# Autodesk Inventor assembly: Assembly
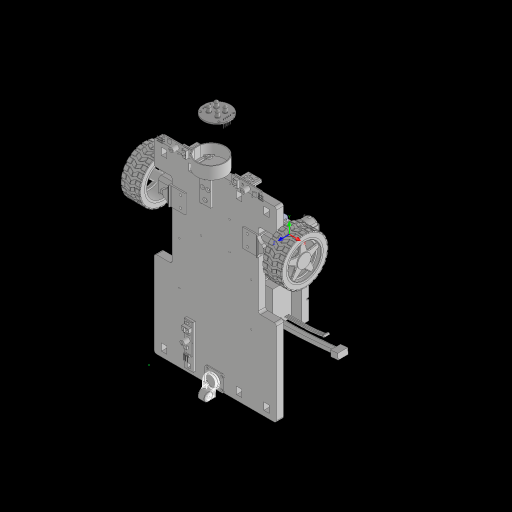
[picture p0: Inventor's stored thumbnail of the model, 512x512]
Saved by Autodesk Inventor 2024.3 (Build 283343010, 343A)
## iProperties
Created: 2025-04-09
Part Number: Assembly
Document SubType Name: Assembly
Designer: Oleg Kelner
Author: Oleg Kelner
## Documents named in this file (21)
- D:\Study\Prototyping\Prototyping-SS25-Team-C4\3DModels\Assembly.iam
- D:\Study\Prototyping\Prototyping-SS25-Team-C4\3DModels\Basic components\chassis.ipt
- D:\Study\Prototyping\Prototyping-SS25-Team-C4\3DModels\Basic components\motor-with-tire.ipt
- D:\Study\Prototyping\Prototyping-SS25-Team-C4\3DModels\Basic components\front-wheel.ipt
- D:\Study\Prototyping\Prototyping-SS25-Team-C4\3DModels\Basic components\motor-with-tire_MIR.ipt
- D:\Study\Prototyping\Prototyping-SS25-Team-C4\3DModels\Basic components\lipo-battery.ipt
- D:\Study\Prototyping\Prototyping-SS25-Team-C4\3DModels\Basic components\arduino.ipt
- D:\Study\Prototyping\Prototyping-SS25-Team-C4\3DModels\Basic components\breadboard.ipt
- D:\Study\Prototyping\Prototyping-SS25-Team-C4\3DModels\Basic components\motorcontroler.ipt
- D:\Study\Prototyping\Prototyping-SS25-Team-C4\3DModels\Details to print\.ipt\vertMotorHolder.ipt
- D:\Study\Prototyping\Prototyping-SS25-Team-C4\3DModels\Details to print\.ipt\batteryHolder.ipt
- D:\Work\HSHL\Kart\Kart Assembly Parts\infrared-sensor-new.ipt
- D:\Study\Prototyping\Prototyping-SS25-Team-C4\3DModels\Details to print\.ipt\IRsensorHolder.ipt
- D:\Study\Prototyping\Prototyping-SS25-Team-C4\3DModels\Details to print\.ipt\IRsensorHolder2.ipt
- D:\Work\HSHL\Kart\Kart Assembly Parts\ultrasonic-sensor.ipt
- D:\Work\HSHL\Kart\Kart Assembly Parts\ColourSensor.ipt
- D:\Study\Prototyping\Prototyping-SS25-Team-C4\3DModels\Details to print\.ipt\ultrasomicHolder.ipt
- D:\Study\Prototyping\Prototyping-SS25-Team-C4\3DModels\Details to print\.ipt\IRHolder_new.ipt
- D:\Study\Prototyping\Prototyping-SS25-Team-C4\3DModels\Details to print\.ipt\IRHolder_new2.ipt
- D:\Study\Prototyping\Prototyping-SS25-Team-C4\3DModels\Details to print\.ipt\colorSensorHolder.ipt
- D:\Study\Prototyping\Prototyping-SS25-Team-C4\3DModels\Details to print\.ipt\colorSensorHolder2.ipt
## Components (26 placed, 20 different names)
1. chassis:1 — Rigid:1, Rigid:2, Rigid:3, Slider:1, Angle:1, Mate:1, Flush:2, Mate:3, Flush:5, Flush:6, Planar:2, Angle:2, Planar:3, Flush:8, Angle:3, Flush:10, Flush:14, Flush:15, Flush:16, Flush:18
2. motor-with-tire:1 — Rotational:11, Rotational:12, Tangent:1
3. front-wheel:1 — Rigid:1
4. motor-with-tire_MIR:1 — Rotational:9, Rotational:10
5. lipo-battery:1 — Slider:1, Rigid:4, Rigid:5, Rigid:6
6. arduino:1 — Planar:2, Angle:2
7. breadboard:1 — Rigid:5
8. motorcontroler:1 — Planar:3, Flush:7, Flush:8
9. vertMotorHolder:1 — Rigid:3, Mate:2, Rotational:11, Rotational:12, Flush:7
10. vertMotorHolder:2 — Rigid:2, Rotational:9, Rotational:10
11. batteryHolder:1 — Mate:2, Rigid:4
12. batteryHolder:2 — Rigid:6
13. infrared-sensor-new:1 — Rotational:5, Rotational:6, Flush:9
14. IRsensorHolder:1 — Angle:1, Rotational:5, Rotational:6, Mate:4, Flush:11
15. IRsensorHolder2:1 — Mate:1, Flush:2, Flush:10, Mate:4, Flush:11
16. infrared-sensor-new:2 — Rotational:7, Rotational:8, Flush:9
17. IRsensorHolder:2 — Rotational:7, Rotational:8, Slider:3
18. IRsensorHolder2:2 — Slider:3, Mate:3, Flush:5, Flush:6
19. ColourSensor:1
20. ultrasonic-sensor:2 — Flush:12, Flush:13
21. ultrasomicHolder:1 — Flush:12, Flush:13
22. IRHolder_new:1 — Flush:14, Flush:15, Rigid:7
23. infrared-sensor-new:3 — Rigid:7
24. IRHolder_new2:1 — Flush:16, Flush:18
25. colorSensorHolder:1 — Flush:19, Flush:20
26. colorSensorHolder2:1 — Flush:19, Flush:20
## Relationships (43: Flush 16, RevoluteJoint 8, WeldJoint 7, Mate 4, Angle 3, TranslationJoint 2, PlanarJoint 2, Tangent 1)
- Rigid:1 [WeldJoint]: chassis:1 ↔ front-wheel:1
- Rigid:2 [WeldJoint] (-30 mm): chassis:1 ↔ vertMotorHolder:2
- Rigid:3 [WeldJoint] (30 mm): chassis:1 ↔ vertMotorHolder:1
- Slider:1 [TranslationJoint]: chassis:1 ↔ lipo-battery:1
- Angle:1 (0 deg): chassis:1 ↔ IRsensorHolder:1
- Rotational:5 [RevoluteJoint]: infrared-sensor-new:1 ↔ IRsensorHolder:1
- Rotational:6 [RevoluteJoint]: infrared-sensor-new:1 ↔ IRsensorHolder:1
- Mate:1: chassis:1 ↔ IRsensorHolder2:1
- Flush:2 (40 mm): chassis:1 ↔ IRsensorHolder2:1
- Mate:2 (30 mm): vertMotorHolder:1 ↔ batteryHolder:1
- Rotational:7 [RevoluteJoint]: infrared-sensor-new:2 ↔ IRsensorHolder:2
- Rotational:8 [RevoluteJoint]: infrared-sensor-new:2 ↔ IRsensorHolder:2
- Slider:3 [TranslationJoint]: IRsensorHolder:2 ↔ IRsensorHolder2:2
- Mate:3: chassis:1 ↔ IRsensorHolder2:2
- Flush:5 (-40 mm): chassis:1 ↔ IRsensorHolder2:2
- Flush:6 (-2.5 mm): chassis:1 ↔ IRsensorHolder2:2
- Rigid:4 [WeldJoint] (-15 mm): lipo-battery:1 ↔ batteryHolder:1
- Rigid:5 [WeldJoint] (2.5 mm): lipo-battery:1 ↔ breadboard:1
- Rotational:9 [RevoluteJoint]: motor-with-tire_MIR:1 ↔ vertMotorHolder:2
- Rotational:10 [RevoluteJoint]: motor-with-tire_MIR:1 ↔ vertMotorHolder:2
- Rotational:11 [RevoluteJoint]: motor-with-tire:1 ↔ vertMotorHolder:1
- Rotational:12 [RevoluteJoint]: motor-with-tire:1 ↔ vertMotorHolder:1
- Rigid:6 [WeldJoint] (-15 mm): lipo-battery:1 ↔ batteryHolder:2
- Planar:2: chassis:1 ↔ arduino:1
- Angle:2 (0 deg): chassis:1 ↔ arduino:1
- Planar:3: chassis:1 ↔ motorcontroler:1
- Flush:7: motorcontroler:1 ↔ vertMotorHolder:1
- Flush:8 (63.3 mm): chassis:1 ↔ motorcontroler:1
- Flush:9: infrared-sensor-new:1 ↔ infrared-sensor-new:2
- Angle:3 (0 deg): chassis:1
- Tangent:1: motor-with-tire:1
- Flush:10 (-2.5 mm): chassis:1 ↔ IRsensorHolder2:1
- Mate:4: IRsensorHolder:1 ↔ IRsensorHolder2:1
- Flush:11: IRsensorHolder:1 ↔ IRsensorHolder2:1
- Flush:12: ultrasonic-sensor:2 ↔ ultrasomicHolder:1
- Flush:13: ultrasonic-sensor:2 ↔ ultrasomicHolder:1
- Flush:14: chassis:1 ↔ IRHolder_new:1
- Flush:15: chassis:1 ↔ IRHolder_new:1
- Rigid:7 [WeldJoint]: IRHolder_new:1 ↔ infrared-sensor-new:3
- Flush:16: chassis:1 ↔ IRHolder_new2:1
- Flush:18: chassis:1 ↔ IRHolder_new2:1
- Flush:19: colorSensorHolder:1 ↔ colorSensorHolder2:1
- Flush:20: colorSensorHolder:1 ↔ colorSensorHolder2:1
## Named parameters: d96_d82 = 0 mm, d97_d83 = 90 deg, d98_d84 = 0 mm, d99_d85 = 180 deg, d100_d91 = 0 mm, d101_d92 = 0.5 mm
